# Autodesk Inventor assembly: ASM Front Drawers
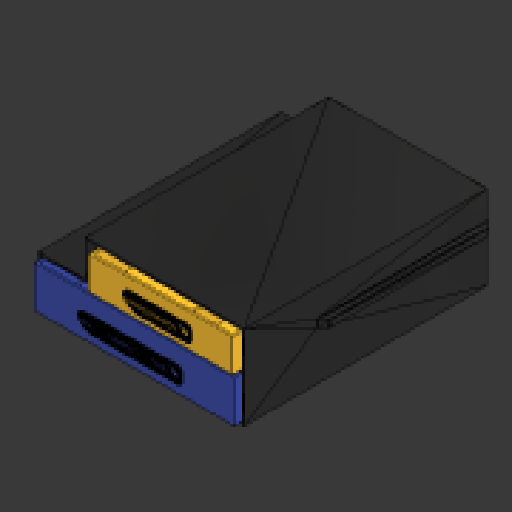
[picture p0: Inventor's stored thumbnail of the model, 512x512]
Saved by Autodesk Inventor 2023 (Build 270158000, 158)
## iProperties
Created: 2023-03-16
Part Number: ASM Front Drawers
Document SubType Name: Assembly
Designer: alber
Author: alber
## Documents named in this file (4)
- C:\Users\alber\Desktop\Files\Ender3-Upgrade\CAD\ASM Front Drawers.iam
- C:\Users\alber\Desktop\Files\Ender3-Upgrade\CAD\CASE.ipt
- C:\Users\alber\Desktop\Files\Ender3-Upgrade\PCB\Ender3 Upgrade\BOTTOM_DRAWER.ipt
- C:\Users\alber\Desktop\Files\Ender3-Upgrade\PCB\Ender3 Upgrade\TOP_DRAWER.ipt
## Components (3 placed, 3 different names)
1. BOTTOM_DRAWER:1 — Mate:2, Mate:3
2. CASE:1 — Mate:1, Mate:2, Mate:3, Mate:4
3. TOP_DRAWER:1 — Mate:1, Mate:4
## Relationships (4: Mate 4)
- Mate:1: CASE:1 ↔ TOP_DRAWER:1
- Mate:2: BOTTOM_DRAWER:1 ↔ CASE:1
- Mate:3: BOTTOM_DRAWER:1 ↔ CASE:1
- Mate:4: CASE:1 ↔ TOP_DRAWER:1
